# Autodesk Inventor assembly: Subframe V1
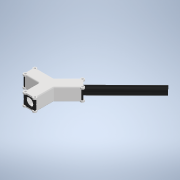
[picture p0: Inventor's stored thumbnail of the model, 180x180]
Saved by Autodesk Inventor 2022 (Build 260153000, 153)
## iProperties
Created: 2022-02-05
Part Number: Subframe V1
Document SubType Name: Assembly
Designer: ultra
Author: ultra
## Documents named in this file (4)
- C:\Users\ultra\Desktop\RAS Aerial\Subframe V1.iam
- C:\Users\ultra\Desktop\RAS Aerial\Tube.ipt
- C:\Users\ultra\Desktop\RAS Aerial\TubeClamp.ipt
- C:\Users\ultra\Desktop\RAS Aerial\BracketV3.ipt
## Components (8 placed, 3 different names)
1. Tube:2 — Insert:4
2. TubeClamp:1 — Flush:5
3. TubeClamp:2 — Flush:5, Insert:2
4. TubeClamp:3 — Flush:6
5. TubeClamp:4 — Insert:3, Flush:6
6. TubeClamp:5 — Angle:1, Insert:1
7. TubeClamp:6
8. BracketV3:1 — Angle:1, Insert:1, Insert:2, Insert:3, Insert:4
## Relationships (10: Flush 5, Insert 4, Angle 1)
- [Flush]: TubeClamp:1 ↔ TubeClamp:2
- [Flush]: TubeClamp:3 ↔ TubeClamp:4
- [Flush]: TubeClamp:5 ↔ TubeClamp:6
- Angle:1 (0 deg): TubeClamp:5 ↔ BracketV3:1
- Insert:1: TubeClamp:5 ↔ BracketV3:1
- Flush:5: TubeClamp:1 ↔ TubeClamp:2
- Insert:2: TubeClamp:2 ↔ BracketV3:1
- Insert:3: TubeClamp:4 ↔ BracketV3:1
- Flush:6: TubeClamp:3 ↔ TubeClamp:4
- Insert:4: Tube:2 ↔ BracketV3:1
## Named parameters: d39_d38 = 0 mm, d43_d39_d38 = 0 mm
